# Autodesk Inventor assembly: コリメータ_エッジフィルター
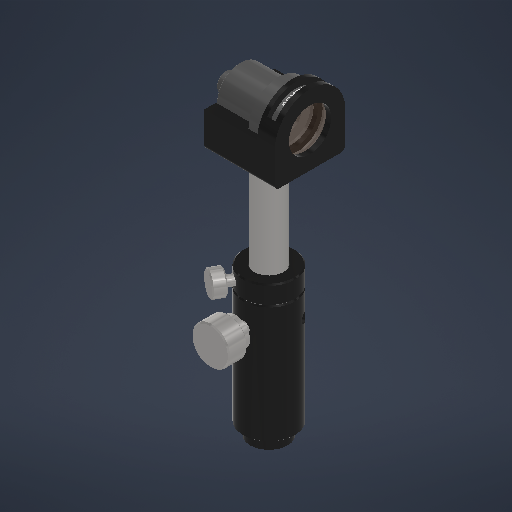
[picture p0: Inventor's stored thumbnail of the model, 512x512]
Saved by Autodesk Inventor 2026 (Build 300175050, 175E)
## iProperties
Created: 2025-07-11
Part Number: コリメータ_エッジフィルター
Document SubType Name: Assembly
Designer: jin20
Author: jin20
## Documents named in this file (6)
- C:\Users\jin20\Documents\装置CAD\RamanSystem\Optics\コリメータ_エッジフィルター.iam
- C:\Users\jin20\Documents\装置CAD\RamanSystem\Optics\コリメータマウント.ipt
- C:\Users\jin20\Documents\装置CAD\RamanSystem\Optics\エッジフィルター.ipt
- C:\Users\jin20\Documents\装置CAD\RamanSystem\Optics\コリメータ.ipt
- C:\Users\jin20\Documents\装置CAD\RamanSystem\Optics\ロッド\ロッド_60mm.ipt
- C:\Users\jin20\Documents\装置CAD\RamanSystem\Optics\ロッドスタンド.ipt
## Components (5 placed, 5 different names)
1. コリメータマウント:1 — 挿入:1, 挿入:2, 挿入:3
2. エッジフィルター:1 — 挿入:1
3. コリメータ:1 — 挿入:2
4. ロッド_60mm:1 — 挿入:3, リジッド:1
5. ロッドスタンド:1 — リジッド:1
## Relationships (4: Insert 3, WeldJoint 1)
- 挿入:1 [Insert]: コリメータマウント:1 ↔ エッジフィルター:1
- 挿入:2 [Insert]: コリメータマウント:1 ↔ コリメータ:1
- 挿入:3 [Insert]: コリメータマウント:1 ↔ ロッド_60mm:1
- リジッド:1 [WeldJoint] (43 mm): ロッド_60mm:1 ↔ ロッドスタンド:1
